# Autodesk Inventor assembly: Roller_Bracket_40mm
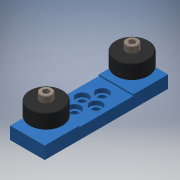
[picture p0: Inventor's stored thumbnail of the model, 180x180]
Saved by Autodesk Inventor 2019.4 (Build 234330000, 330)
## iProperties
Created: 2021-02-01
Part Number: Roller_Bracket_40mm
Document SubType Name: Assembly
Designer: Jorian Brusind
Mass: 44.0669 g
Surface Area: 169.812 cm^2
Volume: 42.4218 cm^3
Density: 1.03878 g/cm^3
Author: Jorian Brusind
## Documents named in this file (4)
- C:\Users\Jorian Brusind\Documents\GitHub\PersonalProjects\HyperRail\Inventor Files\Roller_Bracket_40mm.iam
- C:\Users\Jorian Brusind\Documents\GitHub\PersonalProjects\HyperRail\Inventor Files\Back_Bracket_40mm.ipt
- C:\Users\Jorian Brusind\Documents\GitHub\PersonalProjects\HyperRail\Inventor Files\11mm_BearingWheel.ipt
- C:\Users\Jorian Brusind\Documents\GitHub\PersonalProjects\Inventor Projects\Useful models\Metric bolt\Bolt M5 25mm.ipt
## Components (5 placed, 3 different names)
1. Back_Bracket_40mm:1 — Mate:1, Mate:2, Mate:3, Mate:4
2. 11mm_BearingWheel:1 — Mate:1, Mate:2, Mate:5, Mate:8
3. 11mm_BearingWheel:2 — Mate:3, Mate:4, Mate:6, Mate:7
4. Bolt M5 25mm:1 — Mate:6, Mate:7
5. Bolt M5 25mm:2 — Mate:5, Mate:8
## Relationships (8: Mate 8)
- Mate:1: Back_Bracket_40mm:1 ↔ 11mm_BearingWheel:1
- Mate:2 (5 mm): Back_Bracket_40mm:1 ↔ 11mm_BearingWheel:1
- Mate:3: Back_Bracket_40mm:1 ↔ 11mm_BearingWheel:2
- Mate:4 (5 mm): Back_Bracket_40mm:1 ↔ 11mm_BearingWheel:2
- Mate:5: 11mm_BearingWheel:1 ↔ Bolt M5 25mm:2
- Mate:6: 11mm_BearingWheel:2 ↔ Bolt M5 25mm:1
- Mate:7: 11mm_BearingWheel:2 ↔ Bolt M5 25mm:1
- Mate:8: 11mm_BearingWheel:1 ↔ Bolt M5 25mm:2
